# Autodesk Inventor assembly: Payload-Camera
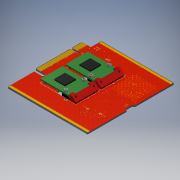
[picture p0: Inventor's stored thumbnail of the model, 180x180]
Saved by Autodesk Inventor 2018 (Build 220112000, 112)
## iProperties
Created: 2019-10-21
Part Number: Payload-Camera
Document SubType Name: Assembly
Designer: Bradley
Author: Bradley
## Documents named in this file (41)
- C:\Users\Bradley\Documents\GitHub\CougSat1-Hardware\CougSat1-Payload\CADModel\Native\Payload-Camera.iam
- C:\Users\Bradley\Documents\GitHub\CougSat1-Hardware\CougSat1-Payload\CADModel\Native\Payload-Camera_PCB.ipt
- C:\Users\Bradley\Documents\GitHub\Resources\SupplierDocuments\26 - Resistor Misc\26-0008\26-0008.ipt
- C:\Users\Bradley\Documents\GitHub\Resources\SupplierDocuments\66 - Sensor\66-0005\66-0005-REV.ipt
- C:\Users\Bradley\Documents\GitHub\Resources\SupplierDocuments\48 - Hardware\48-0078\48-0078.ipt
- C:\Users\Bradley\Documents\GitHub\Resources\SupplierDocuments\48 - Hardware\48-0079\48-0079.ipt
- C:\Users\Bradley\Documents\GitHub\Resources\SupplierDocuments\48 - Hardware\48-0002\48-0002.ipt
- C:\Users\Bradley\Documents\GitHub\Resources\SupplierDocuments\48 - Hardware\48-0240\48-0240.ipt
- C:\Users\Bradley\Documents\GitHub\CougSat1-Hardware\CougSat1-Payload\CADModel\Native\Payload-Camera_Support.ipt
- C:\Users\Bradley\Documents\GitHub\Resources\SupplierDocuments\21 - Resistor 1608\21-0000\21-0000.ipt
- C:\Users\Bradley\Documents\GitHub\Resources\SupplierDocuments\36 - Ferrite\36-152A\36-152A.ipt
- C:\Users\Bradley\Documents\GitHub\Resources\SupplierDocuments\11 - Capacitor Ceramic 1608\11-105B\11-105B.ipt
- C:\Users\Bradley\Documents\GitHub\Resources\SupplierDocuments\11 - Capacitor Ceramic 1608\11-105A\11-105A.ipt
- C:\Users\Bradley\Documents\GitHub\Resources\SupplierDocuments\21 - Resistor 1608\21-1004\21-1004.ipt
- C:\Users\Bradley\Documents\GitHub\Resources\SupplierDocuments\11 - Capacitor Ceramic 1608\11-102A\11-102A.ipt
- C:\Users\Bradley\Documents\GitHub\Resources\SupplierDocuments\21 - Resistor 1608\21-2201\21-2201.ipt
- C:\Users\Bradley\Documents\GitHub\Resources\SupplierDocuments\11 - Capacitor Ceramic 1608\11-2.0A\11-2.0A.ipt
- C:\Users\Bradley\Documents\GitHub\Resources\SupplierDocuments\11 - Capacitor Ceramic 1608\11-4.7A\11-4.7A.ipt
- C:\Users\Bradley\Documents\GitHub\Resources\SupplierDocuments\16 - Capacitor Tantalum SMT\16-475A\16-475A.ipt
- C:\Users\Bradley\Documents\GitHub\Resources\SupplierDocuments\34 - Inductor 3225 and larger\34-472A\34-472A.ipt
- C:\Users\Bradley\Documents\GitHub\Resources\SupplierDocuments\11 - Capacitor Ceramic 1608\11-106A\11-106A.ipt
- C:\Users\Bradley\Documents\GitHub\Resources\SupplierDocuments\21 - Resistor 1608\21-1002\21-1002.ipt
- C:\Users\Bradley\Documents\GitHub\Resources\SupplierDocuments\26 - Resistor Misc\26-0001\26-0001.ipt
- C:\Users\Bradley\Documents\GitHub\Resources\SupplierDocuments\21 - Resistor 1608\21-1005\21-1005.ipt
- C:\Users\Bradley\Documents\GitHub\Resources\SupplierDocuments\11 - Capacitor Ceramic 1608\11-103A\11-103A.ipt
- C:\Users\Bradley\Documents\GitHub\Resources\SupplierDocuments\21 - Resistor 1608\21-2002\21-2002.ipt
- C:\Users\Bradley\Documents\GitHub\Resources\SupplierDocuments\21 - Resistor 1608\21-4702\21-4702.ipt
- C:\Users\Bradley\Documents\GitHub\Resources\SupplierDocuments\21 - Resistor 1608\21-7502\21-7502.ipt
- C:\Users\Bradley\Documents\GitHub\Resources\SupplierDocuments\21 - Resistor 1608\21-1003\21-1003.ipt
- C:\Users\Bradley\Documents\GitHub\Resources\SupplierDocuments\16 - Capacitor Tantalum SMT\16-476A\16-476A.ipt
- C:\Users\Bradley\Documents\GitHub\Resources\SupplierDocuments\11 - Capacitor Ceramic 1608\11-104A\11-104A.ipt
- C:\Users\Bradley\Documents\GitHub\Resources\SupplierDocuments\27 - Conversion IC\27-0003\27-0003.ipt
- C:\Users\Bradley\Documents\GitHub\Resources\SupplierDocuments\08 - Amplifier (excluding RF)\08-0002\08-0002.ipt
- C:\Users\Bradley\Documents\GitHub\Resources\SupplierDocuments\08 - Amplifier (excluding RF)\08-0005\08-0005.ipt
- C:\Users\Bradley\Documents\GitHub\Resources\SupplierDocuments\48 - Hardware\48-0072\48-0072.iam
- C:\Users\Bradley\Documents\GitHub\Resources\SupplierDocuments\28 - Logic IC\28-0004\28-0004.ipt
- C:\Users\Bradley\Documents\GitHub\Resources\SupplierDocuments\27 - Conversion IC\27-0001\27-0001.ipt
- C:\Users\Bradley\Documents\GitHub\Resources\SupplierDocuments\60 - Power IC\60-0007\60-0007.ipt
- C:\Users\Bradley\Documents\GitHub\Resources\SupplierDocuments\60 - Power IC\60-0012\60-0012.ipt
- C:\Users\Bradley\Documents\GitHub\Resources\SupplierDocuments\09 - Communication IC\09-0001\09-0001.ipt
- C:\Users\Bradley\Documents\GitHub\Resources\SupplierDocuments\66 - Sensor\66-0004\66-0004.ipt
## Components (90 placed, 40 different names)
1. 66-0004:1 — Insert:19, Insert:20
2. 09-0001:7 — Mate:167, Mate:178, Mate:179
3. 09-0001:6 — Mate:166, Flush:40, Flush:41
4. 09-0001:5 — Mate:165, Mate:176, Mate:177
5. 09-0001:4 — Mate:164, Mate:174, Mate:175
6. 09-0001:3 — Mate:163, Mate:172, Mate:173
7. 09-0001:2 — Mate:162, Mate:170, Mate:171
8. 09-0001:1 — Mate:161, Mate:168, Mate:169
9. 60-0012:1 — Mate:158, Mate:159, Mate:160
10. 60-0007:1 — Mate:156, Flush:39, Mate:157
11. 27-0001:1 — Mate:154, Mate:155, Flush:38
12. 28-0004:1 — Mate:152, Flush:37, Mate:153
13. 48-0072:1 [sub-assembly] — Mate:151, Mate:180, Flush:42
14. 08-0005:1 — Mate:148, Mate:149, Mate:150
15. 08-0002:2 — Mate:146, Flush:35, Flush:36
16. 08-0002:1 — Mate:145, Flush:34, Mate:147
17. 27-0003:1 — Mate:144, Flush:32, Flush:33
18. 11-104A:16 — Mate:117, Mate:142, Mate:143
19. 11-104A:15 — Mate:116, Mate:140, Mate:141
20. 11-104A:14 — Mate:115, Mate:138, Mate:139
21. 11-104A:13 — Mate:114, Mate:136, Mate:137
22. 11-104A:12 — Mate:113, Mate:134, Mate:135
23. 11-104A:11 — Mate:112, Mate:132, Mate:133
24. 11-104A:10 — Mate:111, Mate:130, Mate:131
25. 11-104A:9 — Mate:110, Mate:128, Mate:129
26. 11-104A:8 — Mate:109, Mate:127, Flush:31
27. 11-104A:7 — Mate:108, Mate:126, Flush:30
28. 11-104A:6 — Mate:107, Mate:125, Flush:29
29. 11-104A:5 — Mate:106, Mate:124, Flush:28
30. 11-104A:4 — Mate:105, Mate:123, Flush:27
31. 11-104A:3 — Mate:104, Mate:121, Mate:122
32. 11-104A:2 — Mate:103, Mate:120, Flush:26
33. 11-104A:1 — Mate:102, Mate:118, Mate:119
34. 16-476A:1 — Mate:99, Mate:100, Mate:101
35. 21-1003:1 — Mate:91, Mate:97, Mate:98
36. 21-7502:1 — Mate:90, Mate:95, Mate:96
37. 21-4702:1 — Mate:89, Mate:93, Mate:94
38. 21-2002:1 — Mate:88, Mate:92, Flush:25
39. 11-103A:1 — Mate:86, Mate:87, Flush:24
40. 21-1005:1 — Mate:83, Mate:84, Mate:85
41. 26-0008:8 — Mate:75, Mate:82, Flush:23
42. 26-0008:7 — Mate:74, Mate:81, Flush:22
43. 26-0008:6 — Mate:73, Mate:80, Flush:21
44. 26-0008:5 — Mate:72, Mate:78, Mate:79
45. 26-0008:4 — Mate:71, Mate:77, Flush:20
46. 26-0008:3 — Mate:70, Mate:76, Flush:19
47. 26-0001:1 — Mate:67, Mate:68, Mate:69
48. 21-1002:3 — Mate:62, Mate:65, Mate:66
49. 21-1002:2 — Mate:61, Mate:64, Flush:18
50. 21-1002:1 — Mate:60, Mate:63, Flush:17
51. 11-106A:5 — Mate:52, Mate:58, Mate:59
52. 11-106A:4 — Mate:51, Mate:57, Flush:16
53. 11-106A:3 — Mate:50, Mate:56, Flush:15
54. 11-106A:2 — Mate:49, Mate:54, Mate:55
55. 11-106A:1 — Mate:48, Mate:53, Flush:14
56. 34-472A:1 — Mate:44, Mate:45, Flush:12
57. 16-475A:1 — Mate:43, Flush:10, Flush:11
58. 11-4.7A:1 — Mate:46, Mate:47, Flush:13
59. 11-2.0A:1 — Mate:41, Mate:42, Flush:9
60. 21-2201:1 — Mate:38, Mate:39, Mate:40
61. 11-102A:1 — Mate:35, Mate:36, Mate:37
62. 21-1004:2 — Mate:30, Mate:31, Mate:32
63. 21-1004:1 — Mate:29, Mate:33, Mate:34
64. 11-105A:2 — Mate:25, Mate:28, Flush:8
65. 11-105A:1 — Mate:24, Mate:26, Mate:27
66. 11-105B:1 — Mate:22, Mate:23, Flush:7
67. 36-152A:1 — Mate:19, Mate:20, Mate:21
68. 21-0000:1 — Mate:7, Mate:11, Mate:12
69. 21-0000:2 — Mate:8, Mate:13, Mate:14
70. 21-0000:3 — Mate:9, Mate:15, Mate:16
71. 21-0000:4 — Mate:10, Mate:17, Mate:18
72. 26-0008:1 — Mate:2, Mate:3, Flush:1
73. 26-0008:2 — Mate:1, Mate:4, Flush:2
74. 48-0002:1 — Insert:1, Insert:2
75. 48-0002:2 — Insert:3, Insert:4
76. 48-0078:1 — Insert:6
77. 48-0079:1 — Insert:5
78. 48-0240:1 — Insert:10
79. 48-0240:2 — Insert:9
80. 48-0240:3 — Insert:8
81. 48-0240:4 — Insert:7
82. 48-0240:5 — Insert:15
83. 48-0240:6 — Insert:16
84. 48-0240:7 — Insert:17
85. 48-0240:8 — Insert:18
86. 66-0005-REV:1 — Mate:5, Flush:3, Flush:4, Insert:1, Insert:2, Insert:5, Insert:9, Insert:10
87. 66-0005-REV:2 — Mate:6, Flush:5, Flush:6, Insert:3, Insert:4, Insert:6, Insert:7, Insert:8
88. Payload-Camera_PCB:1 — Mate:1, Mate:2, Mate:5, Mate:6, Insert:11, Insert:12, Insert:13, Insert:14, Insert:15, Insert:16, Insert:17, Insert:18, Mate:7, Mate:8, Mate:9, Mate:10, Mate:19, Mate:22, Mate:24, Mate:25, Mate:29, Mate:30, Mate:35, Mate:38, Mate:41, Mate:43, Mate:44, Mate:46, Mate:48, Mate:49, Mate:50, Mate:51, Mate:52, Mate:60, Mate:61, Mate:62, Mate:67, Mate:70, Mate:71, Mate:72, Mate:73, Mate:74, Mate:75, Mate:83, Mate:86, Mate:88, Mate:89, Mate:90, Mate:91, Mate:99, Mate:102, Mate:103, Mate:104, Mate:105, Mate:106, Mate:107, Mate:108, Mate:109, Mate:110, Mate:111, Mate:112, Mate:113, Mate:114, Mate:115, Mate:116, Mate:117, Mate:144, Mate:145, Mate:146, Mate:148, Mate:151, Mate:152, Mate:154, Mate:156, Mate:158, Mate:161, Mate:162, Mate:163, Mate:164, Mate:165, Mate:166, Mate:167, Insert:19, Insert:20
89. Payload-Camera_Support:1 — Insert:11, Insert:12
90. Payload-Camera_Support:2 — Insert:13, Insert:14
## Relationships (242: Mate 180, Flush 42, Insert 20)
- Mate:1: 26-0008:2 ↔ Payload-Camera_PCB:1
- Mate:2: 26-0008:1 ↔ Payload-Camera_PCB:1
- Mate:3 (46.5 mm): 26-0008:1
- Flush:1 (-27.75 mm): 26-0008:1
- Mate:4 (46.5 mm): 26-0008:2
- Flush:2 (27.75 mm): 26-0008:2
- Mate:5: 66-0005-REV:1 ↔ Payload-Camera_PCB:1
- Mate:6: 66-0005-REV:2 ↔ Payload-Camera_PCB:1
- Flush:3 (-14 mm): 66-0005-REV:1
- Flush:4 (-33.51 mm): 66-0005-REV:1
- Flush:5 (14 mm): 66-0005-REV:2
- Flush:6 (-33.51 mm): 66-0005-REV:2
- Insert:1: 48-0002:1 ↔ 66-0005-REV:1
- Insert:2: 48-0002:1 ↔ 66-0005-REV:1
- Insert:3: 48-0002:2 ↔ 66-0005-REV:2
- Insert:4: 48-0002:2 ↔ 66-0005-REV:2
- Insert:5: 48-0079:1 ↔ 66-0005-REV:1
- Insert:6: 48-0078:1 ↔ 66-0005-REV:2
- Insert:7: 48-0240:4 ↔ 66-0005-REV:2
- Insert:8: 48-0240:3 ↔ 66-0005-REV:2
- Insert:9: 48-0240:2 ↔ 66-0005-REV:1
- Insert:10: 48-0240:1 ↔ 66-0005-REV:1
- Insert:11: Payload-Camera_PCB:1 ↔ Payload-Camera_Support:1
- Insert:12: Payload-Camera_PCB:1 ↔ Payload-Camera_Support:1
- Insert:13: Payload-Camera_PCB:1 ↔ Payload-Camera_Support:2
- Insert:14: Payload-Camera_PCB:1 ↔ Payload-Camera_Support:2
- Insert:15: 48-0240:5 ↔ Payload-Camera_PCB:1
- Insert:16: 48-0240:6 ↔ Payload-Camera_PCB:1
- Insert:17: 48-0240:7 ↔ Payload-Camera_PCB:1
- Insert:18: 48-0240:8 ↔ Payload-Camera_PCB:1
- Mate:7: 21-0000:1 ↔ Payload-Camera_PCB:1
- Mate:8: 21-0000:2 ↔ Payload-Camera_PCB:1
- Mate:9: 21-0000:3 ↔ Payload-Camera_PCB:1
- Mate:10: 21-0000:4 ↔ Payload-Camera_PCB:1
- Mate:11 (21.7 mm): 21-0000:1
- Mate:12 (11 mm): 21-0000:1
- Mate:13 (21.7 mm): 21-0000:2
- Mate:14 (12.75 mm): 21-0000:2
- Mate:15 (41.75 mm): 21-0000:3
- Mate:16 (21.25 mm): 21-0000:3
- Mate:17 (41.75 mm): 21-0000:4
- Mate:18 (19.5 mm): 21-0000:4
- Mate:19: 36-152A:1 ↔ Payload-Camera_PCB:1
- Mate:20 (11.5 mm): 36-152A:1
- Mate:21 (24.75 mm): 36-152A:1
- Mate:22: 11-105B:1 ↔ Payload-Camera_PCB:1
- Mate:23 (38.75 mm): 11-105B:1
- Flush:7 (-24.75 mm): 11-105B:1
- Mate:24: 11-105A:1 ↔ Payload-Camera_PCB:1
- Mate:25: 11-105A:2 ↔ Payload-Camera_PCB:1
- Mate:26 (77 mm): 11-105A:1
- Mate:27 (-25 mm): 11-105A:1
- Mate:28 (-24.5 mm): 11-105A:2
- Flush:8 (-69.75 mm): 11-105A:2
- Mate:29: 21-1004:1 ↔ Payload-Camera_PCB:1
- Mate:30: 21-1004:2 ↔ Payload-Camera_PCB:1
- Mate:31 (13 mm): 21-1004:2
- Mate:32 (74 mm): 21-1004:2
- Mate:33 (41.75 mm): 21-1004:1
- Mate:34 (23 mm): 21-1004:1
- Mate:35: 11-102A:1 ↔ Payload-Camera_PCB:1
- Mate:36 (79.5 mm): 11-102A:1
- Mate:37 (15.5 mm): 11-102A:1
- Mate:38: 21-2201:1 ↔ Payload-Camera_PCB:1
- Mate:39 (13 mm): 21-2201:1
- Mate:40 (72.25 mm): 21-2201:1
- Mate:41: 11-2.0A:1 ↔ Payload-Camera_PCB:1
- Mate:42 (14.75 mm): 11-2.0A:1
- Flush:9 (-83.75 mm): 11-2.0A:1
- Mate:43: 16-475A:1 ↔ Payload-Camera_PCB:1
- Flush:10 (-28.75 mm): 16-475A:1
- Flush:11 (-11.5 mm): 16-475A:1
- Mate:44: 34-472A:1 ↔ Payload-Camera_PCB:1
- Mate:45 (22.25 mm): 34-472A:1
- Flush:12 (-33 mm): 34-472A:1
- Mate:46: 11-4.7A:1 ↔ Payload-Camera_PCB:1
- Mate:47 (41.75 mm): 11-4.7A:1
- Flush:13 (-24.75 mm): 11-4.7A:1
- Mate:48: 11-106A:1 ↔ Payload-Camera_PCB:1
- Mate:49: 11-106A:2 ↔ Payload-Camera_PCB:1
- Mate:50: 11-106A:3 ↔ Payload-Camera_PCB:1
- Mate:51: 11-106A:4 ↔ Payload-Camera_PCB:1
- Mate:52: 11-106A:5 ↔ Payload-Camera_PCB:1
- Mate:53 (11.75 mm): 11-106A:1
- Flush:14 (-82 mm): 11-106A:1
- Mate:54 (31.25 mm): 11-106A:2
- Mate:55 (36.75 mm): 11-106A:2
- Mate:56 (38.75 mm): 11-106A:3
- Flush:15 (-19.5 mm): 11-106A:3
- Mate:57 (-22.5 mm): 11-106A:4
- Flush:16 (-76.25 mm): 11-106A:4
- Mate:58 (63.35 mm): 11-106A:5
- Mate:59 (24.2 mm): 11-106A:5
- Mate:60: 21-1002:1 ↔ Payload-Camera_PCB:1
- Mate:61: 21-1002:2 ↔ Payload-Camera_PCB:1
- Mate:62: 21-1002:3 ↔ Payload-Camera_PCB:1
- Mate:63 (69.25 mm): 21-1002:1
- Flush:17 (-6.25 mm): 21-1002:1
- Mate:64 (76.5 mm): 21-1002:2
- Flush:18 (-15.5 mm): 21-1002:2
- Mate:65 (23.7 mm): 21-1002:3
- Mate:66 (65.85 mm): 21-1002:3
- Mate:67: 26-0001:1 ↔ Payload-Camera_PCB:1
- Mate:68 (-29.75 mm): 26-0001:1
- Mate:69 (69.75 mm): 26-0001:1
- Mate:70: 26-0008:3 ↔ Payload-Camera_PCB:1
- Mate:71: 26-0008:4 ↔ Payload-Camera_PCB:1
- Mate:72: 26-0008:5 ↔ Payload-Camera_PCB:1
- Mate:73: 26-0008:6 ↔ Payload-Camera_PCB:1
- Mate:74: 26-0008:7 ↔ Payload-Camera_PCB:1
- Mate:75: 26-0008:8 ↔ Payload-Camera_PCB:1
- Mate:76 (-42.5 mm): 26-0008:3
- Flush:19 (-4.25 mm): 26-0008:3
- Mate:77 (-42.47 mm): 26-0008:4
- Flush:20 (-88.04 mm): 26-0008:4
- Mate:78 (28 mm): 26-0008:5
- Mate:79 (36.25 mm): 26-0008:5
- Mate:80 (36.45 mm): 26-0008:6
- Flush:21 (-57 mm): 26-0008:6
- Mate:81 (42.5 mm): 26-0008:7
- Flush:22 (-88 mm): 26-0008:7
- Mate:82 (42.5 mm): 26-0008:8
- Flush:23 (-12.25 mm): 26-0008:8
- Mate:83: 21-1005:1 ↔ Payload-Camera_PCB:1
- Mate:84 (14.75 mm): 21-1005:1
- Mate:85 (82 mm): 21-1005:1
- Mate:86: 11-103A:1 ↔ Payload-Camera_PCB:1
- Mate:87 (39.5 mm): 11-103A:1
- Flush:24 (-34.75 mm): 11-103A:1
- Mate:88: 21-2002:1 ↔ Payload-Camera_PCB:1
- Mate:89: 21-4702:1 ↔ Payload-Camera_PCB:1
- Mate:90: 21-7502:1 ↔ Payload-Camera_PCB:1
- Mate:91: 21-1003:1 ↔ Payload-Camera_PCB:1
- Mate:92 (72.25 mm): 21-2002:1
- Flush:25 (-6.25 mm): 21-2002:1
- Mate:93 (11.75 mm): 21-4702:1
- Mate:94 (83.775 mm): 21-4702:1
- Mate:95 (13 mm): 21-7502:1
- Mate:96 (70.475 mm): 21-7502:1
- Mate:97 (41.75 mm): 21-1003:1
- Mate:98 (17.75 mm): 21-1003:1
- Mate:99: 16-476A:1 ↔ Payload-Camera_PCB:1
- Mate:100 (40 mm): 16-476A:1
- Mate:101 (27.75 mm): 16-476A:1
- Mate:102: 11-104A:1 ↔ Payload-Camera_PCB:1
- Mate:103: 11-104A:2 ↔ Payload-Camera_PCB:1
- Mate:104: 11-104A:3 ↔ Payload-Camera_PCB:1
- Mate:105: 11-104A:4 ↔ Payload-Camera_PCB:1
- Mate:106: 11-104A:5 ↔ Payload-Camera_PCB:1
- Mate:107: 11-104A:6 ↔ Payload-Camera_PCB:1
- Mate:108: 11-104A:7 ↔ Payload-Camera_PCB:1
- Mate:109: 11-104A:8 ↔ Payload-Camera_PCB:1
- Mate:110: 11-104A:9 ↔ Payload-Camera_PCB:1
- Mate:111: 11-104A:10 ↔ Payload-Camera_PCB:1
- Mate:112: 11-104A:11 ↔ Payload-Camera_PCB:1
- Mate:113: 11-104A:12 ↔ Payload-Camera_PCB:1
- Mate:114: 11-104A:13 ↔ Payload-Camera_PCB:1
- Mate:115: 11-104A:14 ↔ Payload-Camera_PCB:1
- Mate:116: 11-104A:15 ↔ Payload-Camera_PCB:1
- Mate:117: 11-104A:16 ↔ Payload-Camera_PCB:1
- Mate:118 (73.5 mm): 11-104A:1
- Mate:119 (15.5 mm): 11-104A:1
- Mate:120 (28.75 mm): 11-104A:2
- Flush:26 (-14.5 mm): 11-104A:2
- Mate:121 (66.8 mm): 11-104A:3
- Mate:122 (15.5 mm): 11-104A:3
- Mate:123 (0.5 mm): 11-104A:4
- Flush:27 (-67 mm): 11-104A:4
- Mate:124 (-6 mm): 11-104A:5
- Flush:28 (-70 mm): 11-104A:5
- Mate:125 (-11.5 mm): 11-104A:6
- Flush:29 (-17.25 mm): 11-104A:6
- Mate:126 (16.5 mm): 11-104A:7
- Flush:30 (-17.25 mm): 11-104A:7
- Mate:127: 11-104A:8
- Flush:31 (-58 mm): 11-104A:8
- Mate:128 (60.25 mm): 11-104A:9
- Mate:129 (2.5 mm): 11-104A:9
- Mate:130 (24.5 mm): 11-104A:10
- Mate:131 (19.75 mm): 11-104A:10
- Mate:132 (24.5 mm): 11-104A:11
- Mate:133 (8.75 mm): 11-104A:11
- Mate:134 (24.5 mm): 11-104A:12
- Mate:135 (-8.25 mm): 11-104A:12
- Mate:136 (24.5 mm): 11-104A:13
- Mate:137 (-19.25 mm): 11-104A:13
- Mate:138 (73.75 mm): 11-104A:14
- Mate:139 (-21 mm): 11-104A:14
- Mate:140 (79.25 mm): 11-104A:15
- Mate:141 (-26.75 mm): 11-104A:15
- Mate:142 (79.25 mm): 11-104A:16
- Mate:143 (-28.5 mm): 11-104A:16
- Mate:144: 27-0003:1 ↔ Payload-Camera_PCB:1
- Flush:32 (-75 mm): 27-0003:1
- Flush:33 (28.75 mm): 27-0003:1
- Mate:145: 08-0002:1 ↔ Payload-Camera_PCB:1
- Mate:146: 08-0002:2 ↔ Payload-Camera_PCB:1
- Flush:34 (24 mm): 08-0002:1
- Mate:147 (73 mm): 08-0002:1
- Flush:35 (-66.57 mm): 08-0002:2
- Flush:36 (-12.24 mm): 08-0002:2
- Mate:148: 08-0005:1 ↔ Payload-Camera_PCB:1
- Mate:149 (78 mm): 08-0005:1
- Mate:150 (12.5 mm): 08-0005:1
- Mate:151: 48-0072:1 ↔ Payload-Camera_PCB:1
- Mate:152: 28-0004:1 ↔ Payload-Camera_PCB:1
- Flush:37 (-0.5 mm): 28-0004:1
- Mate:153 (73.5 mm): 28-0004:1
- Mate:154: 27-0001:1 ↔ Payload-Camera_PCB:1
- Mate:155 (-6.75 mm): 27-0001:1
- Flush:38 (-73.5 mm): 27-0001:1
- Mate:156: 60-0007:1 ↔ Payload-Camera_PCB:1
- Flush:39 (-38.75 mm): 60-0007:1
- Mate:157 (22.125 mm): 60-0007:1
- Mate:158: 60-0012:1 ↔ Payload-Camera_PCB:1
- Mate:159 (31.75 mm): 60-0012:1
- Mate:160 (40 mm): 60-0012:1
- Mate:161: 09-0001:1 ↔ Payload-Camera_PCB:1
- Mate:162: 09-0001:2 ↔ Payload-Camera_PCB:1
- Mate:163: 09-0001:3 ↔ Payload-Camera_PCB:1
- Mate:164: 09-0001:4 ↔ Payload-Camera_PCB:1
- Mate:165: 09-0001:5 ↔ Payload-Camera_PCB:1
- Mate:166: 09-0001:6 ↔ Payload-Camera_PCB:1
- Mate:167: 09-0001:7 ↔ Payload-Camera_PCB:1
- Mate:168 (24.5 mm): 09-0001:1
- Mate:169 (-13.75 mm): 09-0001:1
- Mate:170 (24.5 mm): 09-0001:2
- Mate:171 (-16.75 mm): 09-0001:2
- Mate:172 (24.5 mm): 09-0001:3
- Mate:173 (17.25 mm): 09-0001:3
- Mate:174 (24.5 mm): 09-0001:4
- Mate:175 (14.25 mm): 09-0001:4
- Mate:176 (24.5 mm): 09-0001:5
- Mate:177 (11.25 mm): 09-0001:5
- Flush:40 (-60.25 mm): 09-0001:6
- Flush:41: 09-0001:6
- Mate:178 (24.5 mm): 09-0001:7
- Mate:179 (-10.75 mm): 09-0001:7
- Insert:19: 66-0004:1 ↔ Payload-Camera_PCB:1
- Insert:20: 66-0004:1 ↔ Payload-Camera_PCB:1
- Mate:180 (73.15 mm): 48-0072:1
- Flush:42 (-21.15 mm): 48-0072:1
